# Autodesk Inventor assembly: アームアセンブリ改
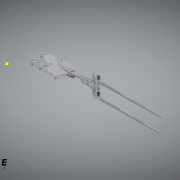
[picture p0: Inventor's stored thumbnail of the model, 180x180]
Saved by Autodesk Inventor 2020 (Build 240168000, 168)
## iProperties
Created: 2020-01-11
Part Number: アームアセンブリ改
Document SubType Name: Assembly
Designer: tanjihayato
Mass: 355.179 g
Surface Area: 2596.72 cm^2
Volume: 225.552 cm^3
Density: 1.57471 g/cm^3
Author: tanjihayato
## Documents named in this file (18)
- \\Mac\Home\Documents\Inventor\2019お遊び機体\アームアセンブリ改.iam
- \\Mac\Home\Documents\Inventor\2019お遊び機体\アームフレーム改２.ipt
- \\Mac\Home\Documents\Inventor\2019お遊び機体\ロッド.ipt
- \\Mac\Home\Documents\Inventor\2019お遊び機体\ロッド根本.ipt
- \\Mac\Home\Documents\Inventor\2019お遊び機体\ロッド根本_MIR.ipt
- \\Mac\Home\Documents\Inventor\2019お遊び機体\ロッド根本２.ipt
- \\Mac\Home\Documents\Inventor\2019お遊び機体\ロッド根本２_MIR.ipt
- \\Mac\Home\Documents\Inventor\2019お遊び機体\アーム中間節.ipt
- \\Mac\Home\Documents\Inventor\2019お遊び機体\アーム中間節_MIR.ipt
- \\Mac\Home\Documents\Inventor\2019お遊び機体\アーム揺動節.ipt
- \\Mac\Home\Documents\Inventor\2019お遊び機体\m2z32.ipt
- \\Mac\Home\Documents\Inventor\2019お遊び機体\スペーサ　m3-l12.ipt
- \\Mac\Home\Documents\Inventor\2019お遊び機体\ツイン抑え.ipt
- \\Mac\Home\Documents\Inventor\2019お遊び機体\ツイン抑え_MIR.ipt
- \\Mac\Home\Documents\Inventor\2019お遊び機体\フランジブッシュ　d6-D8-l5-h12.ipt
- \\Mac\Home\Documents\Inventor\2019お遊び機体\スペーサ　m3-l35.ipt
- \\Mac\Home\Documents\Inventor\プロジェクト名\M1-z10ギア.ipt
- \\Mac\Home\Documents\Inventor\2019お遊び機体\シールド先端.iam
## Components (36 placed, 17 different names)
1. アームフレーム改２:1 — 挿入:1, 挿入:2, 挿入:3, 挿入:4, 挿入:5, 挿入:6, 挿入:7, 挿入:8, 挿入:9, 挿入:10, 挿入:11
2. ロッド:1 — 挿入:29, メイト:9, 挿入:30, メイト:10
3. ロッド根本:1 — 挿入:14, メイト:3, 挿入:16, 挿入:17, 挿入:18
4. ロッド根本_MIR:1 — 挿入:15, メイト:4, 挿入:19, 挿入:20, 挿入:21
5. ロッド根本２:1 — 挿入:24, メイト:7, 挿入:26
6. ロッド根本２_MIR:1 — 挿入:25, メイト:8, 挿入:27
7. ロッド:2 — 挿入:24, メイト:7, 挿入:25, メイト:8
8. アーム中間節:1 — 挿入:13, メイト:1, 挿入:14, メイト:3
9. アーム中間節_MIR:1 — 挿入:12, 挿入:13, メイト:1, メイト:2, 挿入:15, メイト:4, 挿入:34, メイト:11
10. アーム揺動節:1 — 挿入:11, 挿入:12
11. m2z32:1 — 挿入:1, メイト:2
12. スペーサ　m3-l12:1 — 挿入:2
13. スペーサ　m3-l12:2 — 挿入:3
14. スペーサ　m3-l12:3 — 挿入:4
15. スペーサ　m3-l12:4 — 挿入:6
16. スペーサ　m3-l12:5 — 挿入:5
17. スペーサ　m3-l12:6 — 挿入:8
18. スペーサ　m3-l12:7 — 挿入:7
19. スペーサ　m3-l12:8 — 挿入:9
20. スペーサ　m3-l12:9 — 挿入:10
21. スペーサ　m3-l35:1 — 挿入:17, 挿入:23
22. スペーサ　m3-l35:2 — 挿入:18
23. スペーサ　m3-l35:4 — 挿入:21, 挿入:22
24. スペーサ　m3-l35:6 — 挿入:20, メイト:5
25. スペーサ　m3-l35:5 — 挿入:19
26. スペーサ　m3-l35:3 — 挿入:16, メイト:6
27. ロッド根本２:2 — 挿入:29, メイト:9, 挿入:31
28. ロッド根本２_MIR:2 — 挿入:30, メイト:10, 挿入:32
29. ツイン抑え:1 — 挿入:23, メイト:6, 挿入:28
30. ツイン抑え_MIR:1 — 挿入:22, メイト:5, 挿入:33
31. フランジブッシュ　d6-D8-l5-h12:1 — 挿入:26
32. フランジブッシュ　d6-D8-l5-h12:2 — 挿入:27, 挿入:28
33. フランジブッシュ　d6-D8-l5-h12:3 — 挿入:31, 挿入:33
34. フランジブッシュ　d6-D8-l5-h12:4 — 挿入:32
35. M1-z10ギア:1
36. シールド先端:1 [sub-assembly] — 挿入:34, メイト:11
## Relationships (45: Insert 34, Mate 11)
- 挿入:1 [Insert] (1 mm): アームフレーム改２:1 ↔ m2z32:1
- 挿入:2 [Insert]: アームフレーム改２:1 ↔ スペーサ　m3-l12:1
- 挿入:3 [Insert]: アームフレーム改２:1 ↔ スペーサ　m3-l12:2
- 挿入:4 [Insert]: アームフレーム改２:1 ↔ スペーサ　m3-l12:3
- 挿入:5 [Insert]: アームフレーム改２:1 ↔ スペーサ　m3-l12:5
- 挿入:6 [Insert]: アームフレーム改２:1 ↔ スペーサ　m3-l12:4
- 挿入:7 [Insert]: アームフレーム改２:1 ↔ スペーサ　m3-l12:7
- 挿入:8 [Insert]: アームフレーム改２:1 ↔ スペーサ　m3-l12:6
- 挿入:9 [Insert]: アームフレーム改２:1 ↔ スペーサ　m3-l12:8
- 挿入:10 [Insert]: アームフレーム改２:1 ↔ スペーサ　m3-l12:9
- 挿入:11 [Insert] (5 mm): アームフレーム改２:1 ↔ アーム揺動節:1
- 挿入:12 [Insert]: アーム中間節_MIR:1 ↔ アーム揺動節:1
- 挿入:13 [Insert]: アーム中間節:1 ↔ アーム中間節_MIR:1
- メイト:1 [Mate]: アーム中間節:1 ↔ アーム中間節_MIR:1
- メイト:2 [Mate]: アーム中間節_MIR:1 ↔ m2z32:1
- 挿入:14 [Insert]: ロッド根本:1 ↔ アーム中間節:1
- メイト:3 [Mate]: ロッド根本:1 ↔ アーム中間節:1
- 挿入:15 [Insert]: ロッド根本_MIR:1 ↔ アーム中間節_MIR:1
- メイト:4 [Mate]: ロッド根本_MIR:1 ↔ アーム中間節_MIR:1
- 挿入:16 [Insert]: ロッド根本:1 ↔ スペーサ　m3-l35:3
- 挿入:17 [Insert]: ロッド根本:1 ↔ スペーサ　m3-l35:1
- 挿入:18 [Insert]: ロッド根本:1 ↔ スペーサ　m3-l35:2
- 挿入:19 [Insert]: ロッド根本_MIR:1 ↔ スペーサ　m3-l35:5
- 挿入:20 [Insert]: ロッド根本_MIR:1 ↔ スペーサ　m3-l35:6
- 挿入:21 [Insert]: ロッド根本_MIR:1 ↔ スペーサ　m3-l35:4
- 挿入:22 [Insert]: スペーサ　m3-l35:4 ↔ ツイン抑え_MIR:1
- メイト:5 [Mate]: スペーサ　m3-l35:6 ↔ ツイン抑え_MIR:1
- 挿入:23 [Insert]: スペーサ　m3-l35:1 ↔ ツイン抑え:1
- メイト:6 [Mate]: スペーサ　m3-l35:3 ↔ ツイン抑え:1
- 挿入:24 [Insert]: ロッド根本２:1 ↔ ロッド:2
- メイト:7 [Mate]: ロッド根本２:1 ↔ ロッド:2
- 挿入:25 [Insert]: ロッド根本２_MIR:1 ↔ ロッド:2
- メイト:8 [Mate]: ロッド根本２_MIR:1 ↔ ロッド:2
- 挿入:26 [Insert]: ロッド根本２:1 ↔ フランジブッシュ　d6-D8-l5-h12:1
- 挿入:27 [Insert]: ロッド根本２_MIR:1 ↔ フランジブッシュ　d6-D8-l5-h12:2
- 挿入:28 [Insert]: ツイン抑え:1 ↔ フランジブッシュ　d6-D8-l5-h12:2
- 挿入:29 [Insert]: ロッド:1 ↔ ロッド根本２:2
- メイト:9 [Mate]: ロッド:1 ↔ ロッド根本２:2
- 挿入:30 [Insert]: ロッド:1 ↔ ロッド根本２_MIR:2
- メイト:10 [Mate]: ロッド:1 ↔ ロッド根本２_MIR:2
- 挿入:31 [Insert]: ロッド根本２:2 ↔ フランジブッシュ　d6-D8-l5-h12:3
- 挿入:32 [Insert]: ロッド根本２_MIR:2 ↔ フランジブッシュ　d6-D8-l5-h12:4
- 挿入:33 [Insert]: ツイン抑え_MIR:1 ↔ フランジブッシュ　d6-D8-l5-h12:3
- 挿入:34 [Insert]: アーム中間節_MIR:1 ↔ シールド先端:1
- メイト:11 [Mate]: アーム中間節_MIR:1 ↔ シールド先端:1
